# Autodesk Inventor assembly: SPG27_asm
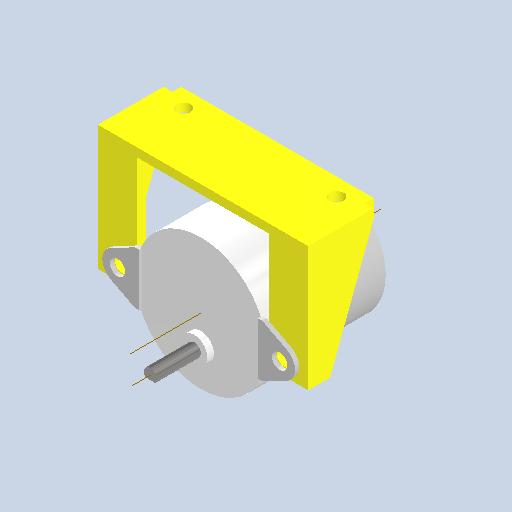
[picture p0: Inventor's stored thumbnail of the model, 512x512]
Saved by Autodesk Inventor 2025.3 (Build 293356030, 356C)
## iProperties
Created: 2025-08-17
Part Number: SPG27_asm
Document SubType Name: Assembly
Designer: daisuke
Author: daisuke
## Documents named in this file (3)
- G:\マイドライブ\project\micro-mouse\3D-Model\SPG27_asm.iam
- G:\マイドライブ\project\micro-mouse\3D-Model\SPG27_Braket.ipt
- G:\マイドライブ\project\micro-mouse\3D-Model\SPG27.ipt
## Components (2 placed, 2 different names)
1. SPG27_Braket:1 — メイト:1, メイト:2, メイト:3
2. SPG27:1 — メイト:1, メイト:2, メイト:3
## Relationships (3: Mate 3)
- メイト:1 [Mate]: SPG27_Braket:1 ↔ SPG27:1
- メイト:2 [Mate]: SPG27_Braket:1 ↔ SPG27:1
- メイト:3 [Mate]: SPG27_Braket:1 ↔ SPG27:1
